# Autodesk Inventor assembly: Assembly9
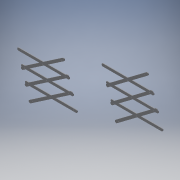
[picture p0: Inventor's stored thumbnail of the model, 180x180]
Saved by Autodesk Inventor 2018 (Build 220112000, 112)
## iProperties
Created: 2018-01-13
Part Number: Assembly9
Document SubType Name: Assembly
Designer: 21alebarron
Author: 21alebarron
## Documents named in this file (2)
- C:\Users\21alebarron\Documents\GitHub\RobotDesigns2018\Assembly9.iam
- H:\DDP\trammel\scissor.ipt
## Components (12 placed, 1 different names)
1. scissor:1 — Mate:1, Mate:2, Mate:7
2. scissor:2 — Mate:1, Mate:2, Mate:3, Mate:6
3. scissor:3 — Mate:3, Mate:6, Mate:8, Mate:9, Mate:17
4. scissor:5 — Mate:7, Mate:8, Mate:9, Mate:12, Mate:13, Mate:14
5. scissor:7 — Mate:15, Mate:16, Mate:17
6. scissor:8 — Mate:12, Mate:13, Mate:14, Mate:15, Mate:16
7. scissor:9
8. scissor:10
9. scissor:11
10. scissor:12
11. scissor:13
12. scissor:14
## Relationships (26: Mate 26)
- Mate:1: scissor:1 ↔ scissor:2
- Mate:2: scissor:1 ↔ scissor:2
- Mate:3: scissor:2 ↔ scissor:3
- Mate:6: scissor:2 ↔ scissor:3
- Mate:7: scissor:1 ↔ scissor:5
- Mate:8: scissor:3 ↔ scissor:5
- Mate:9: scissor:3 ↔ scissor:5
- Mate:12: scissor:5 ↔ scissor:8
- Mate:13: scissor:5 ↔ scissor:8
- Mate:14: scissor:5 ↔ scissor:8
- Mate:15: scissor:7 ↔ scissor:8
- Mate:16: scissor:7 ↔ scissor:8
- Mate:17: scissor:3 ↔ scissor:7
- [Mate]: scissor:9 ↔ scissor:10
- [Mate]: scissor:9 ↔ scissor:10
- [Mate]: scissor:10 ↔ scissor:11
- [Mate]: scissor:10 ↔ scissor:11
- [Mate]: scissor:9 ↔ scissor:12
- [Mate]: scissor:11 ↔ scissor:12
- [Mate]: scissor:11 ↔ scissor:12
- [Mate]: scissor:12 ↔ scissor:14
- [Mate]: scissor:12 ↔ scissor:14
- [Mate]: scissor:12 ↔ scissor:14
- [Mate]: scissor:13 ↔ scissor:14
- [Mate]: scissor:13 ↔ scissor:14
- [Mate]: scissor:11 ↔ scissor:13
## Named parameters: d17_d7 = 0 mm, d18_d8 = 0 mm, d19_d11 = 0 mm, d20_d12 = 0 mm, d21_d13 = 0 mm, d22_d14 = 0 mm, d23_d15 = 0 mm, d24_d16 = 0 mm, d25_d0 = 0 mm, d26_d1 = 0 mm, d27_d2 = 0 mm, d28_d5 = 0 mm, d29_d6 = 0 mm
